# Autodesk Inventor assembly: y-axis
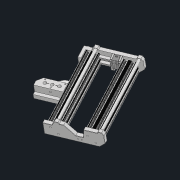
[picture p0: Inventor's stored thumbnail of the model, 180x180]
Saved by Autodesk Inventor 2021 (Build 250183000, 183)
## iProperties
Created: 2021-03-09
Part Number: y-axis
Document SubType Name: Assembly
Designer: Alex
Author: Alex
## Documents named in this file (8)
- C:\Users\arbra\OneDrive\Documents\3D Printer\V1\IPT\ASSEMBLY\y-axis.iam
- C:\Users\arbra\OneDrive\Documents\3D Printer\V1\IPT\PARTS\y-front-V2.ipt
- C:\Users\arbra\OneDrive\Documents\3D Printer\V1\IPT\PARTS\y-idler-V2.ipt
- C:\Users\arbra\OneDrive\Documents\3D Printer\V1\IPT\PARTS\V-Slot 40x40x500 Linear Rail.ipt
- C:\Users\arbra\OneDrive\Documents\3D Printer\V1\IPT\PARTS\y-rear-V2.ipt
- C:\Users\arbra\OneDrive\Documents\3D Printer\V1\IPT\PARTS\Part3.ipt
- C:\Users\arbra\OneDrive\Documents\3D Printer\V1\IPT\PARTS\Part4.ipt
- C:\Users\arbra\OneDrive\Documents\3D Printer\V1\IPT\PARTS\z-bottom.ipt
## Components (8 placed, 7 different names)
1. y-front-V2:1 — Insert:1, Insert:2, Insert:3, Insert:4, Insert:5, Insert:6, Flush:3
2. y-idler-V2:1 — Insert:1, Insert:2
3. V-Slot Linear Rail:1 — Insert:3, Insert:4, Insert:7, Insert:8
4. V-Slot Linear Rail:2 — Insert:5, Insert:6, Insert:9, Insert:10, Mate:1
5. y-rear-V2:1 — Insert:7, Insert:8, Insert:9, Insert:10, Flush:1, Flush:2, Mate:2
6. rod_1 — Flush:1
7. rod_2 — Flush:2
8. z-bottom:1 — Flush:3, Mate:1, Mate:2
## Relationships (15: Insert 10, Flush 3, Mate 2)
- Insert:1: y-front-V2:1 ↔ y-idler-V2:1
- Insert:2: y-front-V2:1 ↔ y-idler-V2:1
- Insert:3: y-front-V2:1 ↔ V-Slot Linear Rail:1
- Insert:4: y-front-V2:1 ↔ V-Slot Linear Rail:1
- Insert:5: y-front-V2:1 ↔ V-Slot Linear Rail:2
- Insert:6: y-front-V2:1 ↔ V-Slot Linear Rail:2
- Insert:7: V-Slot Linear Rail:1 ↔ y-rear-V2:1
- Insert:8: V-Slot Linear Rail:1 ↔ y-rear-V2:1
- Insert:9: V-Slot Linear Rail:2 ↔ y-rear-V2:1
- Insert:10: V-Slot Linear Rail:2 ↔ y-rear-V2:1
- Flush:1: y-rear-V2:1 ↔ rod_1
- Flush:2: y-rear-V2:1 ↔ rod_2
- Flush:3: y-front-V2:1 ↔ z-bottom:1
- Mate:1: V-Slot Linear Rail:2 ↔ z-bottom:1
- Mate:2 (90 mm): y-rear-V2:1 ↔ z-bottom:1
